# Autodesk Inventor assembly: A01 - POV Display Gift Assembly
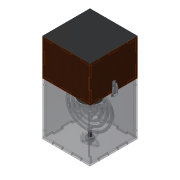
[picture p0: Inventor's stored thumbnail of the model, 180x180]
Saved by Autodesk Inventor 2016 (Build 200138000, 138)
## iProperties
Created: 2016-12-26
Part Number: A01 - POV Display Gift Assembly
Document SubType Name: Conjunto soldado
Designer: Fernando
Weld Material: Aço macio soldado
Mass: 11413.1 g
Surface Area: 12281.4 cm^2
Volume: 4732.62 cm^3
Density: 2.41159 g/cm^3
SurfaceArea_m2: 1.23
Author: Fernando
## Documents named in this file (5)
- G:\00 - Files\00 - Personal\40 - Hobbies\90 - Projetos Particulares\40 - POV Display\01 - Mechanical Design\A01 - POV Display Gift Assembly.iam
- G:\00 - Files\00 - Personal\40 - Hobbies\90 - Projetos Particulares\40 - POV Display\01 - Mechanical Design\A03 - Base Assembly.iam
- G:\00 - Files\00 - Personal\40 - Hobbies\90 - Projetos Particulares\40 - POV Display\01 - Mechanical Design\A04 - Acrylic Visor.iam
- G:\00 - Files\00 - Personal\40 - Hobbies\90 - Projetos Particulares\40 - POV Display\01 - Mechanical Design\P08 - Fecho Rápido.iam
- G:\00 - Files\00 - Personal\40 - Hobbies\90 - Projetos Particulares\40 - POV Display\01 - Mechanical Design\A02_R01 - Main Shaft Assembly.iam
## Components (5 placed, 4 different names)
1. A03 - Base Assembly:1 [sub-assembly] — Mate:1, Flush:1, Flush:2, Flush:3, Flush:5, Insert:5
2. A04 - Acrylic Visor:1 [sub-assembly] — Mate:1, Flush:1, Flush:2, Mate:4, Mate:5
3. P08 - Fecho Rápido:1 [sub-assembly] — Mate:4, Flush:3, Flush:4, Flush:6
4. P08 - Fecho Rápido:2 [sub-assembly] — Mate:5, Flush:5, Flush:6
5. A02_R01 - Main Shaft Assembly:1 [sub-assembly] — Insert:5
## Relationships (10: Flush 6, Mate 3, Insert 1)
- Mate:1: A03 - Base Assembly:1 ↔ A04 - Acrylic Visor:1
- Flush:1: A03 - Base Assembly:1 ↔ A04 - Acrylic Visor:1
- Flush:2: A03 - Base Assembly:1 ↔ A04 - Acrylic Visor:1
- Mate:4: A04 - Acrylic Visor:1 ↔ P08 - Fecho Rápido:1
- Flush:3 (-15 mm): A03 - Base Assembly:1 ↔ P08 - Fecho Rápido:1
- Flush:4: P08 - Fecho Rápido:1
- Mate:5: A04 - Acrylic Visor:1 ↔ P08 - Fecho Rápido:2
- Flush:5 (-15 mm): A03 - Base Assembly:1 ↔ P08 - Fecho Rápido:2
- Flush:6: P08 - Fecho Rápido:1 ↔ P08 - Fecho Rápido:2
- Insert:5: A03 - Base Assembly:1 ↔ A02_R01 - Main Shaft Assembly:1
